# Autodesk Inventor assembly: motor driver support
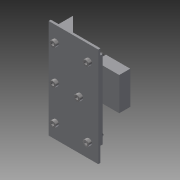
[picture p0: Inventor's stored thumbnail of the model, 180x180]
Saved by Autodesk Inventor 2015 (Build 190159000, 159)
## iProperties
Created: 2015-05-04
Part Number: motor driver support
Document SubType Name: Assembly
Designer: Kuba
Author: Kuba
## Documents named in this file (7)
- C:\Users\Kuba\Dysk Google\synergia\Synergolf\model\GOLF\driver\motor driver support.iam
- C:\Users\Kuba\Dysk Google\synergia\Synergolf\model\GOLF\driver\blacha pionowa.ipt
- C:\Users\Kuba\Dysk Google\synergia\Synergolf\model\GOLF\MostekH.ipt
- C:\Users\Kuba\Dysk Google\synergia\Synergolf\model\GOLF\driver\wspornik.ipt
- C:\Users\Kuba\Dysk Google\synergia\Synergolf\model\GOLF\ContentCenter\pl-PL\DIN 912\DIN 912 - M3 x 0,5 x 12 x 10,75.ipt
- C:\Users\Kuba\Dysk Google\synergia\Synergolf\model\GOLF\ContentCenter\pl-PL\DIN 439-2\DIN 439 - M2,5 x 0,45.ipt
- C:\Users\Kuba\Dysk Google\synergia\Synergolf\model\GOLF\driver\docisk do mostka.ipt
## Components (17 placed, 6 different names)
1. blacha pionowa:1 — Zestawiający:1, Równoległy:1, Równoległy:2, Zestawiający:2, Równoległy:3, Równoległy:4, Równoległy:5, Równoległy:6, Zestawiający:3, Wstaw:1, Wstaw:2, Wstaw:3, Wstaw:4, Wstaw:5, Wstaw:6
2. MostekH:1 — Zestawiający:1, Równoległy:1, Równoległy:2, Wstaw:7, Wstaw:8, Wstaw:9, Wstaw:10, Wstaw:11, Wstaw:12, Zestawiający:4, Równoległy:7, Równoległy:8
3. wspornik:1 — Zestawiający:2, Równoległy:3, Równoległy:4
4. wspornik:2 — Równoległy:5, Równoległy:6, Zestawiający:3
5. DIN 912 - zastąpiona przez DIN EN ISO 4762 M3 x 12:1 — Wstaw:1
6. DIN 912 - zastąpiona przez DIN EN ISO 4762 M3 x 12:2 — Wstaw:2
7. DIN 912 - zastąpiona przez DIN EN ISO 4762 M3 x 12:3 — Wstaw:3
8. DIN 912 - zastąpiona przez DIN EN ISO 4762 M3 x 12:4 — Wstaw:4
9. DIN 912 - zastąpiona przez DIN EN ISO 4762 M3 x 12:5 — Wstaw:5
10. DIN 912 - zastąpiona przez DIN EN ISO 4762 M3 x 12:6 — Wstaw:6
11. DIN 439-2 - zastąpiona przez DIN EN 24035/28675 M2,5:1 — Wstaw:7
12. DIN 439-2 - zastąpiona przez DIN EN 24035/28675 M2,5:2 — Wstaw:8
13. DIN 439-2 - zastąpiona przez DIN EN 24035/28675 M2,5:3 — Wstaw:9
14. DIN 439-2 - zastąpiona przez DIN EN 24035/28675 M2,5:4 — Wstaw:10
15. DIN 439-2 - zastąpiona przez DIN EN 24035/28675 M2,5:5 — Wstaw:11
16. DIN 439-2 - zastąpiona przez DIN EN 24035/28675 M2,5:6 — Wstaw:12
17. docisk do mostka:1 — Zestawiający:4, Równoległy:7, Równoległy:8
## Relationships (24: Insert 12, Flush 8, Mate 4)
- Zestawiający:1 [Mate] (2 mm): blacha pionowa:1 ↔ MostekH:1
- Równoległy:1 [Flush] (2 mm): blacha pionowa:1 ↔ MostekH:1
- Równoległy:2 [Flush]: blacha pionowa:1 ↔ MostekH:1
- Zestawiający:2 [Mate]: blacha pionowa:1 ↔ wspornik:1
- Równoległy:3 [Flush]: blacha pionowa:1 ↔ wspornik:1
- Równoległy:4 [Flush] (7 mm): blacha pionowa:1 ↔ wspornik:1
- Równoległy:5 [Flush]: blacha pionowa:1 ↔ wspornik:2
- Równoległy:6 [Flush] (7 mm): blacha pionowa:1 ↔ wspornik:2
- Zestawiający:3 [Mate]: blacha pionowa:1 ↔ wspornik:2
- Wstaw:1 [Insert]: blacha pionowa:1 ↔ DIN 912 - zastąpiona przez DIN EN ISO 4762 M3 x 12:1
- Wstaw:2 [Insert]: blacha pionowa:1 ↔ DIN 912 - zastąpiona przez DIN EN ISO 4762 M3 x 12:2
- Wstaw:3 [Insert]: blacha pionowa:1 ↔ DIN 912 - zastąpiona przez DIN EN ISO 4762 M3 x 12:3
- Wstaw:4 [Insert]: blacha pionowa:1 ↔ DIN 912 - zastąpiona przez DIN EN ISO 4762 M3 x 12:4
- Wstaw:5 [Insert]: blacha pionowa:1 ↔ DIN 912 - zastąpiona przez DIN EN ISO 4762 M3 x 12:5
- Wstaw:6 [Insert]: blacha pionowa:1 ↔ DIN 912 - zastąpiona przez DIN EN ISO 4762 M3 x 12:6
- Wstaw:7 [Insert]: MostekH:1 ↔ DIN 439-2 - zastąpiona przez DIN EN 24035/28675 M2,5:1
- Wstaw:8 [Insert]: MostekH:1 ↔ DIN 439-2 - zastąpiona przez DIN EN 24035/28675 M2,5:2
- Wstaw:9 [Insert]: MostekH:1 ↔ DIN 439-2 - zastąpiona przez DIN EN 24035/28675 M2,5:3
- Wstaw:10 [Insert]: MostekH:1 ↔ DIN 439-2 - zastąpiona przez DIN EN 24035/28675 M2,5:4
- Wstaw:11 [Insert]: MostekH:1 ↔ DIN 439-2 - zastąpiona przez DIN EN 24035/28675 M2,5:5
- Wstaw:12 [Insert]: MostekH:1 ↔ DIN 439-2 - zastąpiona przez DIN EN 24035/28675 M2,5:6
- Zestawiający:4 [Mate]: MostekH:1 ↔ docisk do mostka:1
- Równoległy:7 [Flush]: MostekH:1 ↔ docisk do mostka:1
- Równoległy:8 [Flush] (0.5 mm): MostekH:1 ↔ docisk do mostka:1
